# Autodesk Inventor assembly: ASY PNS FDS way1
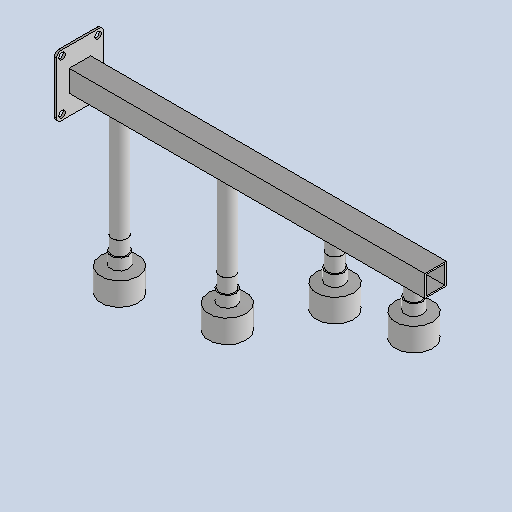
[picture p0: Inventor's stored thumbnail of the model, 512x512]
Saved by Autodesk Inventor 2025 (Build 290162010, 162A)
## iProperties
Created: 2025-07-02
Part Number: ASY PNS FDS way1
Document SubType Name: Assembly
Designer: user
Author: user
## Documents named in this file (8)
- C:\Users\admin\Yandex.Disk\home pc\Inventor\PNS-Panaevsk\Workspace\ASY PNS FDS way1.iam
- C:\Users\admin\Yandex.Disk\home pc\Inventor\PNS-Panaevsk\Workspace\PNS 754 FDS 1200 way tube 1.ipt
- C:\Users\admin\Yandex.Disk\home pc\Inventor\PNS-Panaevsk\PNS dummy filter element.ipt
- C:\Users\admin\Yandex.Disk\home pc\Inventor\PNS-Panaevsk\PNS dummy pipe nippel.ipt
- C:\Users\admin\Yandex.Disk\home pc\Inventor\PNS-Panaevsk\Workspace\PNS 757 FDS 1200 way tube 4.ipt
- C:\Users\admin\Yandex.Disk\home pc\Inventor\PNS-Panaevsk\Workspace\PNS 758 FDS 1200 way tube 6.ipt
- C:\Users\admin\Yandex.Disk\home pc\Inventor\PNS-Panaevsk\Workspace\PNS 759 FDS 1200 way tube 7.ipt
- C:\Users\admin\Yandex.Disk\home pc\Inventor\PNS-Panaevsk\Workspace\PNS 760 FDS 1200 FLANGE 3.ipt
## Components (13 placed, 7 different names)
1. PNS 754 FDS 1200 way tube 1:1
2. PNS dummy filter element:1
3. PNS dummy pipe nippel:1
4. PNS 757 FDS 1200 way tube 4:1
5. PNS dummy filter element:2
6. PNS dummy pipe nippel:2
7. PNS 758 FDS 1200 way tube 6:1
8. PNS dummy filter element:3
9. PNS dummy pipe nippel:3
10. PNS 759 FDS 1200 way tube 7:1
11. PNS dummy filter element:4
12. PNS dummy pipe nippel:4
13. PNS 760 FDS 1200 FLANGE 3:1
## Relationships (12: WeldJoint 12)
- [WeldJoint]: PNS dummy filter element:1 ↔ PNS dummy pipe nippel:1
- [WeldJoint]: PNS 754 FDS 1200 way tube 1:1 ↔ PNS dummy pipe nippel:1
- [WeldJoint]: PNS dummy filter element:2 ↔ PNS dummy pipe nippel:2
- [WeldJoint]: PNS 757 FDS 1200 way tube 4:1 ↔ PNS dummy pipe nippel:2
- [WeldJoint]: PNS 754 FDS 1200 way tube 1:1 ↔ PNS 757 FDS 1200 way tube 4:1
- [WeldJoint]: PNS dummy filter element:3 ↔ PNS dummy pipe nippel:3
- [WeldJoint]: PNS 758 FDS 1200 way tube 6:1 ↔ PNS dummy pipe nippel:3
- [WeldJoint]: PNS dummy filter element:4 ↔ PNS dummy pipe nippel:4
- [WeldJoint]: PNS 759 FDS 1200 way tube 7:1 ↔ PNS dummy pipe nippel:4
- [WeldJoint]: PNS 754 FDS 1200 way tube 1:1 ↔ PNS 758 FDS 1200 way tube 6:1
- [WeldJoint]: PNS 754 FDS 1200 way tube 1:1 ↔ PNS 759 FDS 1200 way tube 7:1
- [WeldJoint] (-2 mm): PNS 754 FDS 1200 way tube 1:1 ↔ PNS 760 FDS 1200 FLANGE 3:1
## Named parameters: d33_d31 = 0 mm, d37_d34_d31 = 0 mm, d43_d40_d37_d34_d31 = 0 mm, d44_d41 = 0 mm, d47_d45_d43_d40_d37_d34_d31 = 0 mm, d48_d46 = 0 mm
